# Autodesk Inventor assembly: wing_assembly
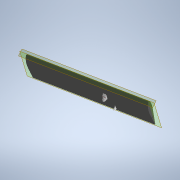
[picture p0: Inventor's stored thumbnail of the model, 180x180]
Saved by Autodesk Inventor 2021 (Build 250183000, 183)
## iProperties
Created: 2020-11-19
Part Number: wing_assembly
Document SubType Name: Assembly
Designer: Paco
Mass: 11.4728 g
Surface Area: 878.625 cm^2
Volume: 368.496 cm^3
Density: 0.031134 g/cm^3
Author: Paco
## Documents named in this file (4)
- C:\Users\victo\Desktop\IISRCAD_BETA2\IISRD_CAD_V_v3\IISRD_V_v2\wing_assembly.iam
- C:\Users\victo\Desktop\IISRCAD_BETA2\IISRD_CAD_V_v3\IISRD_V_v2\IISRD_Wing_Control_surface.ipt
- C:\Users\victo\Desktop\IISRCAD_BETA2\IISRD_CAD_V_v3\IISRD_V_v2\HitecHS40Hitec HS-40 x02.ipt
- C:\Users\victo\Desktop\IISRCAD_BETA2\IISRD_CAD_V_v3\IISRD_V_v2\wing_horn.ipt
## Components (3 placed, 3 different names)
1. IISRD_Wing_v1:1 — Mate:1, Mate:2, Mate:3, Mate:4
2. HitecHS40Hitec HS-40 x02:1 — Mate:1, Mate:2, Mate:3
3. wing_horn:1 — Mate:4
## Relationships (4: Mate 4)
- Mate:1 (-10 mm): IISRD_Wing_v1:1 ↔ HitecHS40Hitec HS-40 x02:1
- Mate:2: IISRD_Wing_v1:1 ↔ HitecHS40Hitec HS-40 x02:1
- Mate:3 (4 mm): IISRD_Wing_v1:1 ↔ HitecHS40Hitec HS-40 x02:1
- Mate:4: IISRD_Wing_v1:1 ↔ wing_horn:1
